# Autodesk Inventor assembly: celestronMountDecHandleAssembly
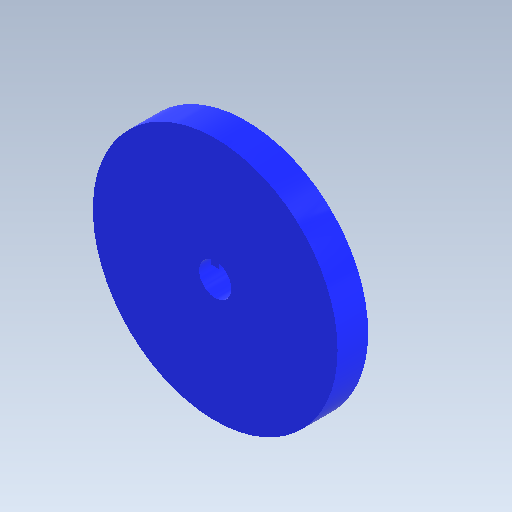
[picture p0: Inventor's stored thumbnail of the model, 512x512]
Saved by Autodesk Inventor 2021.1 (Build 251245010, 245A)
## iProperties
Created: 2020-07-29
Part Number: celestronMountDecHandleAssembly
Document SubType Name: Assembly
Designer: robst
Author: robst
## Documents named in this file (3)
- C:\git\CAD-Development\robSteele\ShapeWays\TelescopeProjects\TelescopeMount\celestronMountDecHandleAssembly.iam
- C:\git\CAD-Development\robSteele\ShapeWays\TelescopeProjects\TelescopeMount\celestronMountDecHandle.ipt
- c:\git\CAD-MfgResources\McMaster-Carr\Insert\10-32x0_310_BRASS HEAT-SET INSERT FOR PLASTIC.ipt
## Components (2 placed, 2 different names)
1. celestronMountDecHandle:1 — Insert:1
2. 10-32x0_310_BRASS HEAT-SET INSERT FOR PLASTIC:1 — Insert:1
## Relationships (1: Insert 1)
- Insert:1: celestronMountDecHandle:1 ↔ 10-32x0_310_BRASS HEAT-SET INSERT FOR PLASTIC:1
